# Autodesk Inventor assembly: Right Side
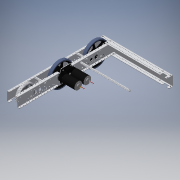
[picture p0: Inventor's stored thumbnail of the model, 180x180]
Saved by Autodesk Inventor 2016 (Build 200138000, 138)
## iProperties
Created: 2016-01-13
Part Number: Right Side
Document SubType Name: Assembly
Designer: Douglas
Author: Douglas
Revision Number: ANY
## Documents named in this file (10)
- D:\SkyDrive\GitHub\2016-Robot-CAD\Inventor\Chassis\Right Side.iam
- D:\SkyDrive\GitHub\2016-Robot-CAD\Inventor\Chassis\AM14U3 Long Frame Half.iam
- D:\SkyDrive\GitHub\2016-Robot-CAD\Inventor\Chassis\am-2598_107 2016 KOP Toughbox Mini.iam
- D:\SkyDrive\GitHub\2016-Robot-CAD\Inventor\Chassis\FR8ZZ Hex Bearing.ipt
- D:\SkyDrive\GitHub\2016-Robot-CAD\Inventor\Chassis\375-16 x 4.25 Hex Bolt_HFBOLT 0.375-16x2.5x1-C.ipt
- D:\SkyDrive\GitHub\2016-Robot-CAD\Inventor\Chassis\375-16 Lock Nut_91831A127.ipt
- D:\SkyDrive\GitHub\2016-Robot-CAD\Inventor\PARTS\x2010-8-FIRSTwheel.iam
- D:\SkyDrive\GitHub\2016-Robot-CAD\Inventor\PARTS\x2010-8-FIRSTwheel-END.iam
- D:\SkyDrive\GitHub\2016-Robot-CAD\Inventor\PARTS\CIM MOTOR AndyMark FR801-001.ipt
- D:\SkyDrive\GitHub\2016-Robot-CAD\Inventor\Chassis\6 HiGrip with bearings, pulleys and spacers.iam
## Components (12 placed, 11 different names)
1. AM14U3 Long Frame Half_3 [sub-assembly] — Mate:12, Mate:14, Mate:15
2. am-2598_107 2016 KOP Toughbox Mini_7 [sub-assembly] — Mate:1, Mate:2, Mate:5, Mate:6, Mate:7, Mate:8, Mate:9, Mate:10
3. FR8ZZ Hex Bearing_8
4. 375-16 x 4.25 Hex Bolt_HFBOLT 0.375-16x2.5x1-C_11 — Mate:11
5. 375-16 x 4.25 Hex Bolt_HFBOLT 0.375-16x2.5x1-C_12 — Mate:13, Mate:14, Mate:15
6. 375-16 Lock Nut_91831A127_13
7. 375-16 Lock Nut_91831A127_14
8. x2010-8-FIRSTwheel:1 [sub-assembly] — Mate:1, Mate:2, Flush:1
9. x2010-8-FIRSTwheel-END:2 [sub-assembly] — Mate:13, Flush:1
10. CIM MOTOR AndyMark FR801-001:1 — Mate:5, Mate:7, Mate:8
11. CIM MOTOR AndyMark FR801-001:2 — Mate:6, Mate:9, Mate:10
12. 6 HiGrip with bearings, pulleys and spacers:1 [sub-assembly] — Mate:11, Mate:12
## Relationships (14: Mate 13, Flush 1)
- Mate:1: am-2598_107 2016 KOP Toughbox Mini_7 ↔ x2010-8-FIRSTwheel:1
- Mate:2: am-2598_107 2016 KOP Toughbox Mini_7 ↔ x2010-8-FIRSTwheel:1
- Mate:5: am-2598_107 2016 KOP Toughbox Mini_7 ↔ CIM MOTOR AndyMark FR801-001:1
- Mate:6: am-2598_107 2016 KOP Toughbox Mini_7 ↔ CIM MOTOR AndyMark FR801-001:2
- Mate:7: am-2598_107 2016 KOP Toughbox Mini_7 ↔ CIM MOTOR AndyMark FR801-001:1
- Mate:8: am-2598_107 2016 KOP Toughbox Mini_7 ↔ CIM MOTOR AndyMark FR801-001:1
- Mate:9: am-2598_107 2016 KOP Toughbox Mini_7 ↔ CIM MOTOR AndyMark FR801-001:2
- Mate:10: am-2598_107 2016 KOP Toughbox Mini_7 ↔ CIM MOTOR AndyMark FR801-001:2
- Mate:11: 375-16 x 4.25 Hex Bolt_HFBOLT 0.375-16x2.5x1-C_11 ↔ 6 HiGrip with bearings, pulleys and spacers:1
- Mate:12: AM14U3 Long Frame Half_3 ↔ 6 HiGrip with bearings, pulleys and spacers:1
- Mate:13: 375-16 x 4.25 Hex Bolt_HFBOLT 0.375-16x2.5x1-C_12 ↔ x2010-8-FIRSTwheel-END:2
- Mate:14: AM14U3 Long Frame Half_3 ↔ 375-16 x 4.25 Hex Bolt_HFBOLT 0.375-16x2.5x1-C_12
- Mate:15: AM14U3 Long Frame Half_3 ↔ 375-16 x 4.25 Hex Bolt_HFBOLT 0.375-16x2.5x1-C_12
- Flush:1: x2010-8-FIRSTwheel:1 ↔ x2010-8-FIRSTwheel-END:2
